# Autodesk Inventor assembly: thin_spacer_box
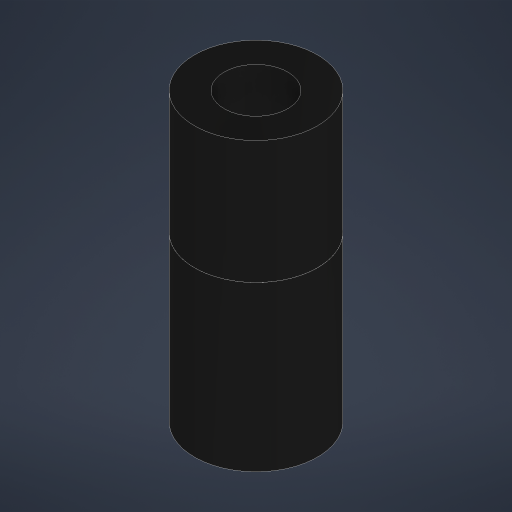
[picture p0: Inventor's stored thumbnail of the model, 512x512]
Saved by Autodesk Inventor 2024 (Build 280153000, 153)
## iProperties
Created: 2023-10-05
Part Number: thin_spacer_box
Document SubType Name: Assembly
Designer: Averey Ku
Author: Averey Ku
## Documents named in this file (4)
- D:\vex_robotics\hardware\cad\VEX-CAD-Inventor-1.41\thin_spacer_box.iam
- D:\vex_robotics\hardware\cad\VEX-CAD-Inventor-1.41\Motion\Spacers\Spacer Nylon .375 OD\NSpacer .375 OD x .375.ipt
- D:\vex_robotics\hardware\cad\VEX-CAD-Inventor-1.41\Motion\Spacers\Spacer Nylon .375 OD.ipt
- D:\vex_robotics\hardware\cad\VEX-CAD-Inventor-1.41\Motion\Spacers\Spacer Nylon .375 OD\NSpacer .375 OD x .500.ipt
## Components (2 placed, 2 different names)
1. NSpacer .375 OD x .375:1 — Insert:1
2. NSpacer .375 OD x .500:2 — Insert:1
## Relationships (1: Insert 1)
- Insert:1: NSpacer .375 OD x .375:1 ↔ NSpacer .375 OD x .500:2
